# Autodesk Inventor assembly: ECE477
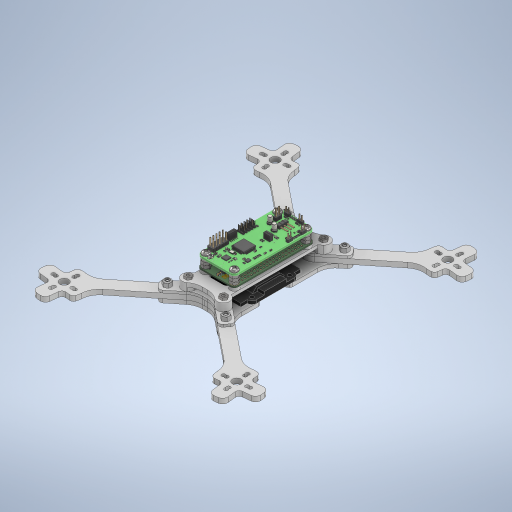
[picture p0: Inventor's stored thumbnail of the model, 512x512]
Saved by Autodesk Inventor 2023 (Build 270158000, 158)
## iProperties
Created: 2022-11-05
Part Number: ECE477
Document SubType Name: Assembly
Designer: mjlangfo
Author: mjlangfo
## Documents named in this file (10)
- C:\Users\Michael\OneDrive - purdue.edu\Senior_Year\Fall_2022\ECE47700\mechanical\ECE477.iam
- C:\Users\Michael\OneDrive - purdue.edu\Senior_Year\Fall_2022\ECE47700\mechanical\Source Two v0.1_import.ipt
- C:\Users\Michael\OneDrive - purdue.edu\Senior_Year\Fall_2022\ECE47700\mechanical\Flight Controller Mount.ipt
- C:\Users\Michael\OneDrive - purdue.edu\Senior_Year\Fall_2022\ECE47700\mechanical\RapberryPiZero.iam
- C:\Users\Michael\OneDrive - purdue.edu\Senior_Year\Fall_2022\ECE47700\mechanical\Velox ESC.ipt
- C:\Users\Michael\OneDrive - purdue.edu\Senior_Year\Fall_2022\ECE47700\mechanical\ECE477_PCB (1).iam
- C:\Users\Michael\Documents\Inventor\Content Center Files\R2023\en-US\AS 1427(08)\AS 1427 - M3 x 5(6) I.ipt
- C:\Users\Michael\Documents\Inventor\Content Center Files\R2023\en-US\NF EN 24036\NF EN 24036 - M2.5.ipt
- C:\Users\Michael\Documents\Inventor\Content Center Files\R2023\en-US\ISO 4032(2)\ISO 4032 - M3 - ISO.ipt
- C:\Users\Michael\Documents\Inventor\Content Center Files\R2023\en-US\SS-ISO 4032\ISO 4032 - M3SS-ISO.ipt
## Components (25 placed, 9 different names)
1. Source Two v0.1_import:1 — Flush:1, Flush:2
2. Flight Controller Mount:1 — Flush:1, Rotational:3, Rotational:4
3. RapberryPiZero:1 [sub-assembly] — Rotational:3, Rotational:4
4. Velox ESC:1 — Flush:2
5. ECE477_PCB (1):1 [sub-assembly]
6. ISO 4032 M3:1
7. SS ISO 4032 M3:1
8. SS ISO 4032 M3:2
9. SS ISO 4032 M3:3
10. SS ISO 4032 M3:4
11. SS ISO 4032 M3:5
12. SS ISO 4032 M3:6
13. SS ISO 4032 M3:7
14. SS ISO 4032 M3:8
15. SS ISO 4032 M3:9
16. SS ISO 4032 M3:10
17. SS ISO 4032 M3:11
18. AS 1427 Z - Metric M3 x 5:5
19. AS 1427 Z - Metric M3 x 5:6
20. AS 1427 Z - Metric M3 x 5:7
21. AS 1427 Z - Metric M3 x 5:8
22. NF EN 24036 M2.5:5
23. NF EN 24036 M2.5:6
24. NF EN 24036 M2.5:7
25. NF EN 24036 M2.5:8
## Relationships (26: Insert 20, RevoluteJoint 4, Flush 2)
- Flush:1: Source Two v0.1_import:1 ↔ Flight Controller Mount:1
- Flush:2: Source Two v0.1_import:1 ↔ Velox ESC:1
- [Insert]: RapberryPiZero:1 ↔ ISO 4032 M3:1
- [Insert]: ISO 4032 M3:1 ↔ SS ISO 4032 M3:1
- [Insert]: SS ISO 4032 M3:1 ↔ SS ISO 4032 M3:2
- [Insert]: RapberryPiZero:1 ↔ SS ISO 4032 M3:3
- [Insert]: SS ISO 4032 M3:3 ↔ SS ISO 4032 M3:4
- [Insert]: SS ISO 4032 M3:4 ↔ SS ISO 4032 M3:5
- [Insert]: RapberryPiZero:1 ↔ SS ISO 4032 M3:6
- [Insert]: SS ISO 4032 M3:6 ↔ SS ISO 4032 M3:7
- [Insert]: SS ISO 4032 M3:7 ↔ SS ISO 4032 M3:8
- [Insert]: RapberryPiZero:1 ↔ SS ISO 4032 M3:9
- [Insert]: SS ISO 4032 M3:9 ↔ SS ISO 4032 M3:10
- [Insert]: SS ISO 4032 M3:10 ↔ SS ISO 4032 M3:11
- [RevoluteJoint]: ECE477_PCB (1):1 ↔ SS ISO 4032 M3:8
- [RevoluteJoint]: ECE477_PCB (1):1 ↔ SS ISO 4032 M3:11
- [Insert]: ECE477_PCB (1):1 ↔ AS 1427 Z - Metric M3 x 5:5
- [Insert]: ECE477_PCB (1):1 ↔ AS 1427 Z - Metric M3 x 5:6
- [Insert]: ECE477_PCB (1):1 ↔ AS 1427 Z - Metric M3 x 5:7
- [Insert]: ECE477_PCB (1):1 ↔ AS 1427 Z - Metric M3 x 5:8
- Rotational:3 [RevoluteJoint]: Flight Controller Mount:1 ↔ RapberryPiZero:1
- Rotational:4 [RevoluteJoint]: Flight Controller Mount:1 ↔ RapberryPiZero:1
- [Insert]: Flight Controller Mount:1 ↔ NF EN 24036 M2.5:5
- [Insert]: Flight Controller Mount:1 ↔ NF EN 24036 M2.5:6
- [Insert]: Flight Controller Mount:1 ↔ NF EN 24036 M2.5:7
- [Insert]: Flight Controller Mount:1 ↔ NF EN 24036 M2.5:8
